# Autodesk Inventor assembly: EnsambleGripper
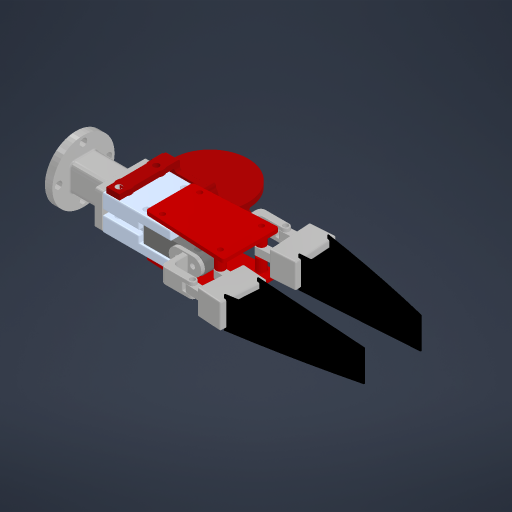
[picture p0: Inventor's stored thumbnail of the model, 512x512]
Saved by Autodesk Inventor 2024.1 (Build 281209000, 209)
## iProperties
Created: 2023-12-07
Part Number: EnsambleGripper
Document SubType Name: Assembly
Designer: Jonathan Leonardo Begambre Rodriguez
Author: Jonathan Leonardo Begambre Rodriguez
## Documents named in this file (4)
- D:\JB\U\20S\1. Roboctic\Laboratory\Robotic-Laboratory-2023-2\Proyecto Final\CAD\EnsambleGripper.iam
- D:\JB\U\20S\1. Roboctic\Laboratory\proyecto\Gripper.ipt
- D:\JB\U\20S\1. Roboctic\Laboratory\Robotic-Laboratory-2023-2\Proyecto Final\CAD\ConectorSoporteVentosa.ipt
- D:\JB\U\20S\1. Roboctic\Laboratory\Robotic-Laboratory-2023-2\Proyecto Final\CAD\SoporteVentosa.ipt
## Components (3 placed, 3 different names)
1. Gripper:1 — Rotational:1
2. ConectorSoporteVentosa:1 — Rotational:1, Mate:1, Mate:2
3. SoporteVentosa:1 — Mate:1, Mate:2
## Relationships (3: Mate 2, RevoluteJoint 1)
- Rotational:1 [RevoluteJoint]: Gripper:1 ↔ ConectorSoporteVentosa:1
- Mate:1: ConectorSoporteVentosa:1 ↔ SoporteVentosa:1
- Mate:2: ConectorSoporteVentosa:1 ↔ SoporteVentosa:1
